# Autodesk Inventor assembly: PeerVavle
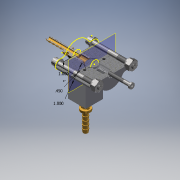
[picture p0: Inventor's stored thumbnail of the model, 180x180]
Saved by Autodesk Inventor 2018 (Build 220112000, 112)
## iProperties
Created: 2020-03-28
Part Number: PeerVavle
Document SubType Name: Assembly
Designer: emile
Author: emile
## Documents named in this file (9)
- C:\Users\emile\OneDrive\Documents\Inventor\Respirator\Peep\AirPressure\PeerVavle.iam
- C:\Users\emile\OneDrive\Documents\Inventor\Respirator\Peep\AirPressure\PeerIntput.ipt
- C:\Users\emile\OneDrive\Documents\Inventor\Respirator\Peep\AirPressure\output.ipt
- C:\Users\emile\OneDrive\Documents\Inventor\Respirator\Peep\9657K810_COMPRESSION SPRING.ipt
- C:\Users\emile\OneDrive\Documents\Inventor\Respirator\Peep\AirPressure\Food-Grade Abrasion-Resistant Natural Rubber Ball 5-8 in.ipt
- C:\Users\emile\OneDrive\Documents\Inventor\Respirator\Peep\9555K330_FOOD-AND-BEVERAGE O-RING.ipt
- C:\Users\emile\OneDrive\Documents\Inventor\Respirator\Peep\AirPressure\Brass Barbed Hose Fitting for Air and Water.ipt
- C:\Users\emile\OneDrive\Documents\Inventor\Respirator\Peep\AirPressure\PeerVavle\Design Accelerator\Bolted Connection1.iam
- C:\Users\emile\OneDrive\Documents\Inventor\Respirator\Peep\AirPressure\PeerVavle\Design Accelerator\Bolted Connection2.iam
## Components (9 placed, 7 different names)
1. PeerIntput:1 — Mate:4, Mate:9, Mate:11, Mate:12, Mate:13, Mate:14, Mate:15, Mate:18, Mate:19
2. output:1 — Mate:1, Mate:3, Flush:1, Mate:5, Mate:6, Tangent:1, Mate:9, Mate:15, Mate:16, Flush:2, Mate:21, Flush:3
3. 9657K810_COMPRESSION SPRING:1 — Mate:1, Mate:5
4. Food-Grade Abrasion-Resistant Natural Rubber Ball 5-8 in:1 — Mate:16, Mate:17
5. 9555K330_FOOD-AND-BEVERAGE O-RING:1 — Mate:6, Tangent:1
6. Brass Barbed Hose Fitting for Air and Water:1 — Mate:11, Mate:12
7. Bolted Connection:1 [sub-assembly] — Mate:13, Mate:14
8. Brass Barbed Hose Fitting for Air and Water:2 — Mate:18, Mate:19
9. Bolted Connection:2 [sub-assembly] — Mate:21, Flush:3
## Relationships (20: Mate 16, Flush 3, Tangent 1)
- Mate:1: output:1 ↔ 9657K810_COMPRESSION SPRING:1
- Mate:3: output:1
- Mate:4: PeerIntput:1
- Flush:1: output:1
- Mate:5: output:1 ↔ 9657K810_COMPRESSION SPRING:1
- Mate:6: output:1 ↔ 9555K330_FOOD-AND-BEVERAGE O-RING:1
- Tangent:1: output:1 ↔ 9555K330_FOOD-AND-BEVERAGE O-RING:1
- Mate:9: PeerIntput:1 ↔ output:1
- Mate:11: PeerIntput:1 ↔ Brass Barbed Hose Fitting for Air and Water:1
- Mate:12: PeerIntput:1 ↔ Brass Barbed Hose Fitting for Air and Water:1
- Mate:13: PeerIntput:1 ↔ Bolted Connection:1
- Mate:14: PeerIntput:1 ↔ Bolted Connection:1
- Mate:15: PeerIntput:1 ↔ output:1
- Mate:16: output:1 ↔ Food-Grade Abrasion-Resistant Natural Rubber Ball 5-8 in:1
- Flush:2 (3.4925 mm): output:1
- Mate:17: Food-Grade Abrasion-Resistant Natural Rubber Ball 5-8 in:1
- Mate:18: PeerIntput:1 ↔ Brass Barbed Hose Fitting for Air and Water:2
- Mate:19: PeerIntput:1 ↔ Brass Barbed Hose Fitting for Air and Water:2
- Mate:21: output:1 ↔ Bolted Connection:2
- Flush:3: output:1 ↔ Bolted Connection:2
